# Autodesk Inventor assembly: Ultrasonic Sensor - Mounted (Right)
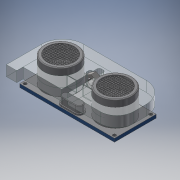
[picture p0: Inventor's stored thumbnail of the model, 180x180]
Saved by Autodesk Inventor 2019.4 (Build 234330000, 330)
## iProperties
Created: 2022-08-15
Part Number: Ultrasonic Sensor - Mounted (Right)
Document SubType Name: Assembly
Designer: Mike Angus
Author: Mike Angus
## Documents named in this file (4)
- O:\User_MA\TSS\MSc IR\CAD\Ultrasonic Sensor - Mounted (Right).iam
- O:\User_MA\TSS\MSc IR\CAD\Ultrasonic Sensor Clamp.ipt
- O:\User_MA\TSS\MSc IR\CAD\HC-SR04-UltrasonicSensor v7.ipt
- O:\User_MA\TSS\MSc IR\CAD\m3Nut.ipt
## Components (3 placed, 3 different names)
1. Ultrasonic Sensor Clamp:1 — Mate:1, Angle:1, Flush:1, Mate:2, Insert:1, Angle:2
2. HC-SR04-UltrasonicSensor v7:1 — Insert:1, Angle:2
3. m3Nut:1 — Mate:1, Angle:1, Flush:1, Mate:2
## Relationships (6: Mate 2, Angle 2, Flush 1, Insert 1)
- Mate:1: Ultrasonic Sensor Clamp:1 ↔ m3Nut:1
- Angle:1 (0 deg): Ultrasonic Sensor Clamp:1 ↔ m3Nut:1
- Flush:1 (22.3 mm): Ultrasonic Sensor Clamp:1 ↔ m3Nut:1
- Mate:2 (-5.6175 mm): Ultrasonic Sensor Clamp:1 ↔ m3Nut:1
- Insert:1 (-7.9 mm): Ultrasonic Sensor Clamp:1 ↔ HC-SR04-UltrasonicSensor v7:1
- Angle:2 (0 deg): Ultrasonic Sensor Clamp:1 ↔ HC-SR04-UltrasonicSensor v7:1
## Named parameters: totalWidth = 50 mm, m3Nut_diam = 5.4 mm
